# Autodesk Inventor assembly: MPG Assy
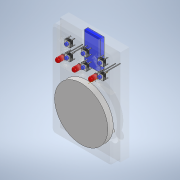
[picture p0: Inventor's stored thumbnail of the model, 180x180]
Saved by Autodesk Inventor 2022 (Build 260153000, 153)
## iProperties
Created: 2022-10-09
Part Number: MPG Assy
Document SubType Name: Assembly
Designer: Nick
Author: Nick
## Documents named in this file (7)
- Y:\Projects\CNC_MPG\MPG Assy.iam
- Y:\Projects\CNC_MPG\Arduino Pro Micro.ipt
- Y:\Projects\CNC_MPG\Button.ipt
- Y:\Projects\CNC_MPG\Case Back.ipt
- Y:\Projects\CNC_MPG\Case Front.ipt
- Y:\Projects\CNC_MPG\MPG.ipt
- Y:\Projects\CNC_MPG\LED.ipt
## Components (13 placed, 6 different names)
1. Arduino Pro Micro:1 — Mate:2, Mate:3
2. Case Front:1 — Insert:1, Insert:2, Insert:3, Insert:4, Insert:5, Insert:6, Insert:7, Insert:8, Insert:9, Insert:10, Mate:1, Flush:1, Flush:2
3. MPG:1 — Insert:1
4. Button:4 — Insert:2
5. Button:5 — Insert:3
6. Button:6 — Insert:5
7. Button:7 — Insert:6
8. Button:8 — Insert:4
9. Button:9 — Insert:7
10. LED:1 — Insert:8
11. LED:2 — Insert:9
12. LED:3 — Insert:10
13. Case Back:1 — Mate:1, Flush:1, Flush:2, Mate:2, Mate:3
## Relationships (15: Insert 10, Mate 3, Flush 2)
- Insert:1: Case Front:1 ↔ MPG:1
- Insert:2: Case Front:1 ↔ Button:4
- Insert:3: Case Front:1 ↔ Button:5
- Insert:4: Case Front:1 ↔ Button:8
- Insert:5: Case Front:1 ↔ Button:6
- Insert:6: Case Front:1 ↔ Button:7
- Insert:7: Case Front:1 ↔ Button:9
- Insert:8: Case Front:1 ↔ LED:1
- Insert:9: Case Front:1 ↔ LED:2
- Insert:10: Case Front:1 ↔ LED:3
- Mate:1: Case Front:1 ↔ Case Back:1
- Flush:1: Case Front:1 ↔ Case Back:1
- Flush:2: Case Front:1 ↔ Case Back:1
- Mate:2: Arduino Pro Micro:1 ↔ Case Back:1
- Mate:3: Arduino Pro Micro:1 ↔ Case Back:1
